# Autodesk Inventor assembly: supports
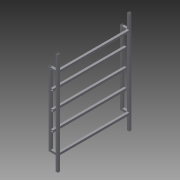
[picture p0: Inventor's stored thumbnail of the model, 180x180]
Saved by Autodesk Inventor 2013 (Build 170138000, 138)
## iProperties
Created: 2012-10-21
Part Number: supports
Document SubType Name: Weldment
Designer: Istvan
Weld Material: Welded Aluminum-6061
Author: Istvan
## Documents named in this file (6)
- D:\GitHub\Crown-Fire\CAD\Frame\Supports\supports.iam
- D:\GitHub\Crown-Fire\CAD\Frame\Supports\tableBrace-fb.ipt
- D:\GitHub\Crown-Fire\CAD\Templates\squareTube_1.5.ipt
- D:\GitHub\Crown-Fire\CAD\Frame\Supports\tableBrace-l.ipt
- D:\GitHub\Crown-Fire\CAD\Frame\Supports\tableBraceStandoff.ipt
- D:\GitHub\Crown-Fire\CAD\Frame\Supports\tableRack.ipt
## Components (13 placed, 4 different names)
1. tableBrace-fb:1 — Mate:4, Flush:8, Flush:9, Flush:21, Flush:22, Mate:21
2. tableBrace-fb:2 — Mate:3, Flush:3, Flush:6, Flush:12, Flush:21, Flush:22, Flush:24, Flush:26
3. tableBrace-l:4 — Mate:3, Mate:4, Flush:3, Mate:6, Mate:7, Mate:8, Mate:9, Flush:5, Flush:7
4. tableBraceStandoff:5 — Mate:9, Flush:12, Mate:17, Flush:25
5. tableBraceStandoff:6 — Mate:6, Flush:7, Flush:8, Mate:10, Flush:15, Flush:16
6. tableBraceStandoff:7 — Mate:7, Flush:9, Flush:23
7. tableBraceStandoff:8 — Mate:8, Flush:5, Flush:6, Mate:11, Flush:13, Flush:14, Mate:20, Flush:26
8. tableRack:9 — Mate:11, Flush:13, Flush:14, Mate:14, Mate:15, Flush:17, Flush:18, Flush:20, Mate:16
9. tableRack:10 — Mate:10, Flush:15, Flush:16, Flush:23
10. tableRack:11 — Flush:20, Mate:16, Mate:18, Mate:19
11. tableRack:12 — Mate:14, Flush:18, Mate:19, Mate:20
12. tableRack:13 — Mate:15, Flush:17, Mate:17, Mate:18
13. tableBrace-l:14 — Mate:21, Flush:24, Flush:25
## Relationships (36: Flush 20, Mate 16)
- Mate:3: tableBrace-fb:2 ↔ tableBrace-l:4
- Mate:4: tableBrace-fb:1 ↔ tableBrace-l:4
- Flush:3: tableBrace-fb:2 ↔ tableBrace-l:4
- Mate:6: tableBrace-l:4 ↔ tableBraceStandoff:6
- Mate:7: tableBrace-l:4 ↔ tableBraceStandoff:7
- Mate:8: tableBrace-l:4 ↔ tableBraceStandoff:8
- Mate:9: tableBrace-l:4 ↔ tableBraceStandoff:5
- Flush:5: tableBrace-l:4 ↔ tableBraceStandoff:8
- Flush:6: tableBrace-fb:2 ↔ tableBraceStandoff:8
- Flush:7: tableBrace-l:4 ↔ tableBraceStandoff:6
- Flush:8: tableBrace-fb:1 ↔ tableBraceStandoff:6
- Flush:9: tableBrace-fb:1 ↔ tableBraceStandoff:7
- Flush:12: tableBrace-fb:2 ↔ tableBraceStandoff:5
- Mate:10: tableBraceStandoff:6 ↔ tableRack:10
- Mate:11: tableBraceStandoff:8 ↔ tableRack:9
- Flush:13: tableBraceStandoff:8 ↔ tableRack:9
- Flush:14: tableBraceStandoff:8 ↔ tableRack:9
- Flush:15: tableBraceStandoff:6 ↔ tableRack:10
- Flush:16: tableBraceStandoff:6 ↔ tableRack:10
- Mate:14: tableRack:9 ↔ tableRack:12
- Mate:15: tableRack:9 ↔ tableRack:13
- Flush:17: tableRack:9 ↔ tableRack:13
- Flush:18: tableRack:9 ↔ tableRack:12
- Flush:20: tableRack:9 ↔ tableRack:11
- Mate:16: tableRack:9 ↔ tableRack:11
- Mate:17 (282.575 mm): tableBraceStandoff:5 ↔ tableRack:13
- Mate:18 (282.575 mm): tableRack:11 ↔ tableRack:13
- Mate:19 (282.575 mm): tableRack:11 ↔ tableRack:12
- Flush:21: tableBrace-fb:1 ↔ tableBrace-fb:2
- Flush:22: tableBrace-fb:1 ↔ tableBrace-fb:2
- Mate:20 (282.575 mm): tableBraceStandoff:8 ↔ tableRack:12
- Flush:23: tableBraceStandoff:7 ↔ tableRack:10
- Mate:21: tableBrace-fb:1 ↔ tableBrace-l:14
- Flush:24: tableBrace-fb:2 ↔ tableBrace-l:14
- Flush:25: tableBraceStandoff:5 ↔ tableBrace-l:14
- Flush:26 (254 mm): tableBrace-fb:2 ↔ tableBraceStandoff:8
